# Autodesk Inventor assembly: Assembly
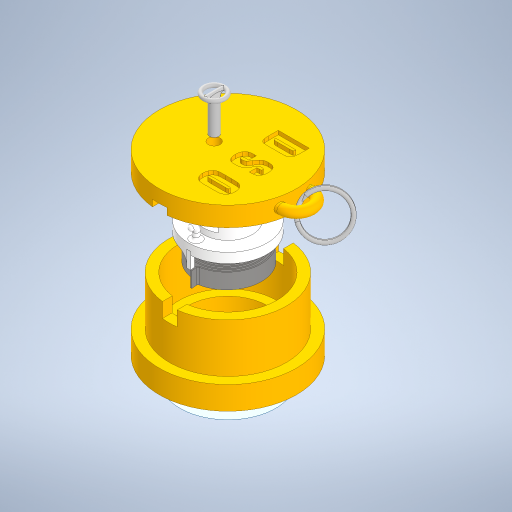
[picture p0: Inventor's stored thumbnail of the model, 512x512]
Saved by Autodesk Inventor 2023 (Build 270158000, 158)
## iProperties
Created: 2022-04-28
Part Number: Assembly
Document SubType Name: Assembly
Designer: AggyT
Author: AggyT
## Documents named in this file (9)
- C:\Users\AggyT\Desktop\College\Undergraduate Archives\Year 2\Spring 2022\ME263\Project Model\Assembly.iam
- C:\Users\AggyT\Desktop\College\Undergraduate Archives\Year 2\Spring 2022\ME263\Project Model\LidBottom.ipt
- C:\Users\AggyT\Desktop\College\Undergraduate Archives\Year 2\Spring 2022\ME263\Project Model\Pin.ipt
- C:\Users\AggyT\Desktop\College\Undergraduate Archives\Year 2\Spring 2022\ME263\Project Model\Top Cap.ipt
- C:\Users\AggyT\Desktop\College\Undergraduate Archives\Year 2\Spring 2022\ME263\Project Model\Wheel.ipt
- C:\Users\AggyT\Desktop\College\Undergraduate Archives\Year 2\Spring 2022\ME263\Project Model\Power Spring.ipt
- C:\Users\AggyT\Desktop\College\Undergraduate Archives\Year 2\Spring 2022\ME263\Project Model\Key Ring.ipt
- C:\Users\AggyT\Desktop\College\Undergraduate Archives\Year 2\Spring 2022\ME263\Project Model\Suction Cup.ipt
- C:\Users\AggyT\Desktop\College\Undergraduate Archives\Year 2\Spring 2022\ME263\Project Model\skf_bearing_624-z_2.iam
## Components (8 placed, 8 different names)
1. LidBottom:1 — Mate:4, Mate:5
2. Pin:1 — Mate:2
3. Top Cap:1 — Mate:1, Mate:2
4. Wheel:1 — Mate:1, Mate:3, Mate:4
5. Power Spring:1
6. Key Ring:1
7. Suction Cup:1 — Mate:5
8. skf_bearing_624-z_2:1 [sub-assembly] — Mate:3
## Relationships (5: Mate 5)
- Mate:1: Top Cap:1 ↔ Wheel:1
- Mate:2: Pin:1 ↔ Top Cap:1
- Mate:3: Wheel:1 ↔ skf_bearing_624-z_2:1
- Mate:4: LidBottom:1 ↔ Wheel:1
- Mate:5: LidBottom:1 ↔ Suction Cup:1
